# Autodesk Inventor assembly: main room, doors, corridor connected
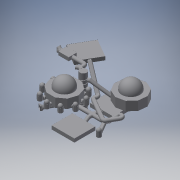
[picture p0: Inventor's stored thumbnail of the model, 180x180]
Saved by Autodesk Inventor 2017 (Build 210142000, 142)
## iProperties
Created: 2018-03-04
Part Number: main room, doors, corridor connected
Document SubType Name: Assembly
Designer: Braxton
Author: Braxton
## Documents named in this file (20)
- E:\School\Game develpment\geoscape\done\single wall\map (one wall)\main room, doors, corridor connected (one wall).iam
- D:\School\Game develpment\geoscape\done (one wall)\rooms  (one wall)\assembly\main room with double door.iam
- E:\School\Game develpment\geoscape\done\single wall\corridors (one wall done)\corridor (one wall).ipt
- E:\School\Game develpment\geoscape\done\single wall\corridors (one wall done)\corridor turn (one wall).ipt
- E:\School\Game develpment\geoscape\done\single wall\corridors (one wall done)\Y corridor  (one wall).ipt
- E:\School\Game develpment\geoscape\done\single wall\corridors (one wall done)\end cap (one wall).ipt
- E:\School\Game develpment\geoscape\done\single wall\corridors (one wall done)\curve ramp (one wall).ipt
- E:\School\Game develpment\geoscape\done\single wall\corridors (one wall done)\ramp top connect  (one wall).ipt
- E:\School\Game develpment\geoscape\done\single wall\corridors (one wall done)\ramp (one wall).ipt
- E:\School\Game develpment\geoscape\done\single wall\corridors (one wall done)\ramp bottom connect (one wall).ipt
- D:\School\Game develpment\geoscape\done (one wall)\rooms  (one wall)\assembly\assembly of dome with corridors with all doors.iam
- E:\School\Game develpment\geoscape\done\single wall\corridors (one wall done)\X corridor  (one wall).ipt
- E:\School\Game develpment\geoscape\done\single wall\corridors (one wall done)\ramp connect both ends  (one wall).ipt
- E:\School\Game develpment\geoscape\done\single wall\rooms  (one wall)\room with 15 cubicals (one wall).ipt
- E:\School\Game develpment\geoscape\done\single wall\rooms  (one wall)\starting room (one wall).ipt
- E:\School\Game develpment\geoscape\done\single wall\doors (one wall)\9 foot door (one wall)\end door room (one wall) (9).ipt
- E:\School\Game develpment\geoscape\done\single wall\rooms  (one wall)\dome  (one wall).ipt
- E:\School\Game develpment\geoscape\done\single wall\rooms  (one wall)\dome with corridors  (one wall).ipt
- E:\School\Game develpment\geoscape\done\single wall\rooms  (one wall)\dome one terminal  (one wall).ipt
- E:\School\Game develpment\geoscape\done\single wall\doors (one wall)\9 foot door (one wall)\(closed face) end door room (one wall) (9).ipt
## Components (70 placed, 19 different names)
1. (closed face) end door room (one wall) (9):1 — Insert:96, Flush:64
2. corridor (one wall):19 — Flush:52, Insert:66, Flush:53, Insert:81, Insert:95, Mate:27
3. corridor (one wall):18 — Flush:51, Flush:52, Insert:65, Insert:66
4. corridor (one wall):17 — Flush:50, Flush:51, Insert:64, Insert:65
5. corridor (one wall):16 — Flush:49, Flush:50, Insert:63, Insert:64
6. corridor (one wall):15 — Flush:48, Flush:49, Insert:62, Insert:63
7. corridor turn (one wall):8 — Mate:14, Flush:48, Insert:61, Insert:62
8. ramp top connect  (one wall):3 — Flush:47, Insert:57, Insert:60, Mate:11
9. ramp (one wall):8 — Flush:46, Flush:47, Insert:56, Insert:57
10. ramp (one wall):7 — Flush:45, Flush:46, Insert:55, Insert:56
11. ramp (one wall):6 — Flush:44, Flush:45, Insert:54, Insert:55
12. ramp (one wall):5 — Flush:43, Flush:44, Insert:53, Insert:54
13. ramp (one wall):4 — Flush:42, Flush:43, Insert:52, Insert:53
14. ramp bottom connect (one wall):3 — Insert:51, Flush:42, Insert:52
15. corridor turn (one wall):7 — Insert:49, Flush:41, Insert:51
16. corridor turn (one wall):6 — Insert:49, Insert:50, Flush:40, Flush:41
17. corridor (one wall):14 — Flush:36, Insert:48, Insert:50, Flush:40
18. corridor (one wall):13 — Flush:36, Flush:37, Insert:47, Insert:48
19. corridor (one wall):12 — Flush:37, Flush:38, Insert:46, Insert:47
20. corridor (one wall):11 — Flush:38, Flush:39, Insert:45, Insert:46
21. corridor (one wall):10 — Flush:39, Insert:44, Insert:45
22. corridor turn (one wall):5 — Flush:34, Insert:42, Insert:44
23. corridor (one wall):9 — Flush:33, Flush:34, Insert:41, Insert:42
24. corridor (one wall):8 — Flush:32, Flush:33, Insert:40, Insert:41
25. corridor turn (one wall):4 — Flush:31, Flush:32, Insert:39, Insert:40
26. corridor turn (one wall):3 — Flush:30, Flush:31, Insert:38, Insert:39
27. ramp top connect  (one wall):2 — Insert:37, Flush:29, Flush:30, Insert:38
28. ramp bottom connect (one wall):2 — Insert:37, Flush:29, Insert:43, Flush:35
29. corridor (one wall):7 — Insert:35, Flush:28, Insert:84, Mate:26
30. corridor (one wall):6 — Insert:34, Insert:35, Flush:27, Flush:28
31. Y corridor  (one wall):2 — Insert:33, Flush:26, Insert:34, Flush:27, Insert:43, Flush:35
32. corridor (one wall):5 — Insert:32, Insert:33, Flush:25, Flush:26
33. ramp connect both ends  (one wall):2 — Insert:30, Flush:24, Insert:58, Mate:12
34. ramp connect both ends  (one wall):1 — Insert:29, Flush:23, Insert:59, Mate:13
35. X corridor  (one wall):1 — Insert:28, Insert:29, Insert:30, Flush:22, Flush:23, Flush:24, Insert:32, Flush:25
36. corridor (one wall):4 — Insert:27, Insert:28, Flush:21, Flush:22
37. corridor (one wall):3 — Insert:26, Insert:27, Flush:20, Flush:21
38. corridor turn (one wall):2 — Insert:26, Insert:31, Mate:9, Flush:20
39. end cap (one wall):3 — Insert:25, Mate:8
40. end cap (one wall):2 — Insert:24, Mate:7
41. ramp bottom connect (one wall):1 — Insert:12, Flush:9, Insert:82, Mate:25
42. ramp (one wall):3 — Insert:11, Flush:8, Insert:12, Flush:9
43. ramp (one wall):2 — Insert:10, Insert:11, Flush:7, Flush:8
44. ramp (one wall):1 — Insert:9, Insert:10, Flush:6, Flush:7
45. ramp top connect  (one wall):1 — Insert:8, Mate:5, Insert:9, Flush:6
46. curve ramp (one wall):1 — Insert:7, Mate:4, Insert:8, Mate:5, Flush:10, Insert:24, Mate:7, Insert:25, Mate:8, Insert:31, Mate:9, Mate:14, Insert:61, Insert:77, Insert:83, Flush:54
47. end cap (one wall):1 — Insert:6, Flush:5
48. Y corridor  (one wall):1 — Insert:5, Flush:4, Insert:6, Flush:5, Insert:7, Mate:4
49. corridor turn (one wall):1 — Insert:4, Flush:3, Insert:5, Flush:4
50. corridor (one wall):2 — Insert:3, Flush:2, Insert:4, Flush:3
51. corridor (one wall):1 — Insert:2, Insert:3, Mate:3, Flush:2, Mate:19, Insert:79
52. end door room (one wall) (9):2 — Flush:53, Insert:81, Insert:95, Mate:27
53. starting room (one wall):1 — Mate:19, Insert:79, Insert:96, Flush:64
54. room with 15 cubicals (one wall):1 — Insert:58, Mate:12
55. room with 15 cubicals (one wall):2 — Insert:59, Mate:13
56. room with 15 cubicals (one wall):3 — Insert:60, Mate:11
57. assembly of dome with corridors with all doors:1 [sub-assembly] — Flush:10, Insert:77
58. main room with double door:1 [sub-assembly] — Insert:2, Mate:3
59. dome  (one wall):1 — Insert:82, Mate:25
60. dome with corridors  (one wall):1 — Insert:83, Flush:54, Insert:85, Insert:86, Insert:87, Insert:88, Insert:89, Insert:90, Insert:91, Insert:92, Insert:93, Flush:55, Flush:56, Flush:57, Flush:58, Flush:59, Flush:60, Flush:61, Flush:62, Flush:63
61. dome one terminal  (one wall):1 — Insert:84, Mate:26
62. dome one terminal  (one wall):2 — Insert:85, Flush:55
63. dome one terminal  (one wall):3 — Insert:86, Flush:56
64. dome one terminal  (one wall):4 — Insert:87, Flush:57
65. dome one terminal  (one wall):5 — Insert:88, Flush:58
66. dome one terminal  (one wall):6 — Insert:89, Flush:59
67. dome one terminal  (one wall):7 — Insert:90, Flush:60
68. dome one terminal  (one wall):8 — Insert:91, Flush:61
69. dome one terminal  (one wall):9 — Insert:92, Flush:62
70. dome one terminal  (one wall):10 — Insert:93, Flush:63
## Relationships (138: Insert 70, Flush 54, Mate 14)
- Insert:2: corridor (one wall):1 ↔ main room with double door:1
- Insert:3: corridor (one wall):2 ↔ corridor (one wall):1
- Mate:3: corridor (one wall):1 ↔ main room with double door:1
- Flush:2: corridor (one wall):2 ↔ corridor (one wall):1
- Insert:4: corridor turn (one wall):1 ↔ corridor (one wall):2
- Flush:3: corridor turn (one wall):1 ↔ corridor (one wall):2
- Insert:5: Y corridor  (one wall):1 ↔ corridor turn (one wall):1
- Flush:4: Y corridor  (one wall):1 ↔ corridor turn (one wall):1
- Insert:6: end cap (one wall):1 ↔ Y corridor  (one wall):1
- Flush:5: end cap (one wall):1 ↔ Y corridor  (one wall):1
- Insert:7: curve ramp (one wall):1 ↔ Y corridor  (one wall):1
- Mate:4: curve ramp (one wall):1 ↔ Y corridor  (one wall):1
- Insert:8: ramp top connect  (one wall):1 ↔ curve ramp (one wall):1
- Mate:5: ramp top connect  (one wall):1 ↔ curve ramp (one wall):1
- Insert:9: ramp (one wall):1 ↔ ramp top connect  (one wall):1
- Insert:10: ramp (one wall):2 ↔ ramp (one wall):1
- Insert:11: ramp (one wall):3 ↔ ramp (one wall):2
- Flush:6: ramp (one wall):1 ↔ ramp top connect  (one wall):1
- Flush:7: ramp (one wall):2 ↔ ramp (one wall):1
- Flush:8: ramp (one wall):3 ↔ ramp (one wall):2
- Insert:12: ramp bottom connect (one wall):1 ↔ ramp (one wall):3
- Flush:9: ramp bottom connect (one wall):1 ↔ ramp (one wall):3
- Flush:10: curve ramp (one wall):1 ↔ assembly of dome with corridors with all doors:1
- Insert:24: end cap (one wall):2 ↔ curve ramp (one wall):1
- Mate:7: end cap (one wall):2 ↔ curve ramp (one wall):1
- Insert:25: end cap (one wall):3 ↔ curve ramp (one wall):1
- Mate:8: end cap (one wall):3 ↔ curve ramp (one wall):1
- Insert:26: corridor (one wall):3 ↔ corridor turn (one wall):2
- Insert:27: corridor (one wall):4 ↔ corridor (one wall):3
- Insert:28: X corridor  (one wall):1 ↔ corridor (one wall):4
- Insert:29: ramp connect both ends  (one wall):1 ↔ X corridor  (one wall):1
- Insert:30: ramp connect both ends  (one wall):2 ↔ X corridor  (one wall):1
- Insert:31: corridor turn (one wall):2 ↔ curve ramp (one wall):1
- Mate:9: corridor turn (one wall):2 ↔ curve ramp (one wall):1
- Flush:20: corridor (one wall):3 ↔ corridor turn (one wall):2
- Flush:21: corridor (one wall):4 ↔ corridor (one wall):3
- Flush:22: X corridor  (one wall):1 ↔ corridor (one wall):4
- Flush:23: ramp connect both ends  (one wall):1 ↔ X corridor  (one wall):1
- Flush:24: ramp connect both ends  (one wall):2 ↔ X corridor  (one wall):1
- Insert:32: corridor (one wall):5 ↔ X corridor  (one wall):1
- Insert:33: Y corridor  (one wall):2 ↔ corridor (one wall):5
- Flush:25: corridor (one wall):5 ↔ X corridor  (one wall):1
- Flush:26: Y corridor  (one wall):2 ↔ corridor (one wall):5
- Insert:34: corridor (one wall):6 ↔ Y corridor  (one wall):2
- Insert:35: corridor (one wall):7 ↔ corridor (one wall):6
- Flush:27: corridor (one wall):6 ↔ Y corridor  (one wall):2
- Flush:28: corridor (one wall):7 ↔ corridor (one wall):6
- Insert:37: ramp top connect  (one wall):2 ↔ ramp bottom connect (one wall):2
- Flush:29: ramp top connect  (one wall):2 ↔ ramp bottom connect (one wall):2
- Flush:30: corridor turn (one wall):3 ↔ ramp top connect  (one wall):2
- Flush:31: corridor turn (one wall):4 ↔ corridor turn (one wall):3
- Flush:32: corridor (one wall):8 ↔ corridor turn (one wall):4
- Flush:33: corridor (one wall):9 ↔ corridor (one wall):8
- Flush:34: corridor turn (one wall):5 ↔ corridor (one wall):9
- Insert:38: corridor turn (one wall):3 ↔ ramp top connect  (one wall):2
- Insert:39: corridor turn (one wall):4 ↔ corridor turn (one wall):3
- Insert:40: corridor (one wall):8 ↔ corridor turn (one wall):4
- Insert:41: corridor (one wall):9 ↔ corridor (one wall):8
- Insert:42: corridor turn (one wall):5 ↔ corridor (one wall):9
- Insert:43: ramp bottom connect (one wall):2 ↔ Y corridor  (one wall):2
- Flush:35: ramp bottom connect (one wall):2 ↔ Y corridor  (one wall):2
- Flush:36: corridor (one wall):14 ↔ corridor (one wall):13
- Flush:37: corridor (one wall):13 ↔ corridor (one wall):12
- Flush:38: corridor (one wall):12 ↔ corridor (one wall):11
- Flush:39: corridor (one wall):11 ↔ corridor (one wall):10
- Insert:44: corridor (one wall):10 ↔ corridor turn (one wall):5
- Insert:45: corridor (one wall):11 ↔ corridor (one wall):10
- Insert:46: corridor (one wall):12 ↔ corridor (one wall):11
- Insert:47: corridor (one wall):13 ↔ corridor (one wall):12
- Insert:48: corridor (one wall):14 ↔ corridor (one wall):13
- Insert:49: corridor turn (one wall):7 ↔ corridor turn (one wall):6
- Insert:50: corridor turn (one wall):6 ↔ corridor (one wall):14
- Flush:40: corridor turn (one wall):6 ↔ corridor (one wall):14
- Flush:41: corridor turn (one wall):7 ↔ corridor turn (one wall):6
- Insert:51: ramp bottom connect (one wall):3 ↔ corridor turn (one wall):7
- Flush:42: ramp (one wall):4 ↔ ramp bottom connect (one wall):3
- Flush:43: ramp (one wall):5 ↔ ramp (one wall):4
- Flush:44: ramp (one wall):6 ↔ ramp (one wall):5
- Flush:45: ramp (one wall):7 ↔ ramp (one wall):6
- Flush:46: ramp (one wall):8 ↔ ramp (one wall):7
- Flush:47: ramp top connect  (one wall):3 ↔ ramp (one wall):8
- Insert:52: ramp (one wall):4 ↔ ramp bottom connect (one wall):3
- Insert:53: ramp (one wall):5 ↔ ramp (one wall):4
- Insert:54: ramp (one wall):6 ↔ ramp (one wall):5
- Insert:55: ramp (one wall):7 ↔ ramp (one wall):6
- Insert:56: ramp (one wall):8 ↔ ramp (one wall):7
- Insert:57: ramp top connect  (one wall):3 ↔ ramp (one wall):8
- Insert:58: ramp connect both ends  (one wall):2 ↔ room with 15 cubicals (one wall):1
- Insert:59: ramp connect both ends  (one wall):1 ↔ room with 15 cubicals (one wall):2
- Insert:60: ramp top connect  (one wall):3 ↔ room with 15 cubicals (one wall):3
- Mate:11: ramp top connect  (one wall):3 ↔ room with 15 cubicals (one wall):3
- Mate:12: ramp connect both ends  (one wall):2 ↔ room with 15 cubicals (one wall):1
- Mate:13: ramp connect both ends  (one wall):1 ↔ room with 15 cubicals (one wall):2
- Mate:14: corridor turn (one wall):8 ↔ curve ramp (one wall):1
- Flush:48: corridor (one wall):15 ↔ corridor turn (one wall):8
- Flush:49: corridor (one wall):16 ↔ corridor (one wall):15
- Flush:50: corridor (one wall):17 ↔ corridor (one wall):16
- Flush:51: corridor (one wall):18 ↔ corridor (one wall):17
- Flush:52: corridor (one wall):19 ↔ corridor (one wall):18
- Insert:61: corridor turn (one wall):8 ↔ curve ramp (one wall):1
- Insert:62: corridor (one wall):15 ↔ corridor turn (one wall):8
- Insert:63: corridor (one wall):16 ↔ corridor (one wall):15
- Insert:64: corridor (one wall):17 ↔ corridor (one wall):16
- Insert:65: corridor (one wall):18 ↔ corridor (one wall):17
- Insert:66: corridor (one wall):19 ↔ corridor (one wall):18
- Insert:77: curve ramp (one wall):1 ↔ assembly of dome with corridors with all doors:1
- Mate:19: corridor (one wall):1 ↔ starting room (one wall):1
- Insert:79: corridor (one wall):1 ↔ starting room (one wall):1
- Flush:53: corridor (one wall):19 ↔ end door room (one wall) (9):2
- Insert:81: corridor (one wall):19 ↔ end door room (one wall) (9):2
- Insert:82: ramp bottom connect (one wall):1 ↔ dome  (one wall):1
- Mate:25: ramp bottom connect (one wall):1 ↔ dome  (one wall):1
- Insert:83: curve ramp (one wall):1 ↔ dome with corridors  (one wall):1
- Flush:54: curve ramp (one wall):1 ↔ dome with corridors  (one wall):1
- Insert:84: corridor (one wall):7 ↔ dome one terminal  (one wall):1
- Insert:85: dome with corridors  (one wall):1 ↔ dome one terminal  (one wall):2
- Insert:86: dome with corridors  (one wall):1 ↔ dome one terminal  (one wall):3
- Insert:87: dome with corridors  (one wall):1 ↔ dome one terminal  (one wall):4
- Insert:88: dome with corridors  (one wall):1 ↔ dome one terminal  (one wall):5
- Insert:89: dome with corridors  (one wall):1 ↔ dome one terminal  (one wall):6
- Insert:90: dome with corridors  (one wall):1 ↔ dome one terminal  (one wall):7
- Insert:91: dome with corridors  (one wall):1 ↔ dome one terminal  (one wall):8
- Insert:92: dome with corridors  (one wall):1 ↔ dome one terminal  (one wall):9
- Insert:93: dome with corridors  (one wall):1 ↔ dome one terminal  (one wall):10
- Flush:55: dome with corridors  (one wall):1 ↔ dome one terminal  (one wall):2
- Flush:56: dome with corridors  (one wall):1 ↔ dome one terminal  (one wall):3
- Flush:57: dome with corridors  (one wall):1 ↔ dome one terminal  (one wall):4
- Flush:58: dome with corridors  (one wall):1 ↔ dome one terminal  (one wall):5
- Flush:59: dome with corridors  (one wall):1 ↔ dome one terminal  (one wall):6
- Flush:60: dome with corridors  (one wall):1 ↔ dome one terminal  (one wall):7
- Flush:61: dome with corridors  (one wall):1 ↔ dome one terminal  (one wall):8
- Flush:62: dome with corridors  (one wall):1 ↔ dome one terminal  (one wall):9
- Flush:63: dome with corridors  (one wall):1 ↔ dome one terminal  (one wall):10
- Mate:26: corridor (one wall):7 ↔ dome one terminal  (one wall):1
- Insert:95: corridor (one wall):19 ↔ end door room (one wall) (9):2
- Mate:27: corridor (one wall):19 ↔ end door room (one wall) (9):2
- Insert:96: (closed face) end door room (one wall) (9):1 ↔ starting room (one wall):1
- Flush:64: (closed face) end door room (one wall) (9):1 ↔ starting room (one wall):1
